# Autodesk Inventor assembly: lift block assy
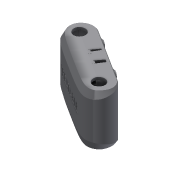
[picture p0: Inventor's stored thumbnail of the model, 180x180]
Saved by Autodesk Inventor 2016 (Build 200138000, 138)
## iProperties
Created: 2016-08-18
Part Number: lift block assy
Document SubType Name: Assembly
Designer: admin
Author: admin
## Documents named in this file (9)
- C:\Users\admin\Desktop\creatablaeD3-이준영 인수인계\1612 3D 도면\lift block assy\lift block assy.iam
- C:\Users\admin\Desktop\creatablaeD3-이준영 인수인계\1612 3D 도면\lift block assy\ball_bushing.ipt
- C:\Users\admin\Desktop\creatablaeD3-이준영 인수인계\1612 3D 도면\lift block assy\belt_fixer.ipt
- C:\Users\admin\Desktop\creatablaeD3-이준영 인수인계\1612 3D 도면\lift block assy\lift_block_cover_back.ipt
- C:\Users\admin\Desktop\creatablaeD3-이준영 인수인계\1612 3D 도면\lift block assy\lift_block_cover_front.ipt
- C:\Users\admin\Desktop\creatablaeD3-이준영 인수인계\1612 3D 도면\lift block assy\m4 15 flat_head_socket.ipt
- C:\Users\admin\Desktop\creatablaeD3-이준영 인수인계\1612 3D 도면\lift block assy\magnet.ipt
- C:\Users\admin\Desktop\creatablaeD3-이준영 인수인계\1612 3D 도면\lift block assy\Ms3 8 BH_tapping_screw.ipt
- C:\Users\admin\Desktop\creatablaeD3-이준영 인수인계\1612 3D 도면\lift block assy\nut_M4.ipt
## Components (13 placed, 8 different names)
1. ball_bushing:1 — Mate:4, Mate:6
2. belt_fixer:1 — Mate:1, Mate:2
3. lift_block_cover_back:1 — Mate:1, Mate:2, Mate:3, Mate:4, Mate:5, Mate:8
4. lift_block_cover_front:1 — Mate:6, Mate:7, Mate:8
5. m4 15 flat_head_socket:1 — Rotational:1, Mate:3
6. magnet:1
7. Ms3 8 BH_tapping_screw:1
8. nut_M4:1 — Rotational:1
9. ball_bushing:2 — Mate:5, Mate:7
10. magnet:2
11. Ms3 8 BH_tapping_screw:2
12. Ms3 8 BH_tapping_screw:3
13. Ms3 8 BH_tapping_screw:4
## Relationships (9: Mate 8, RevoluteJoint 1)
- Mate:1: belt_fixer:1 ↔ lift_block_cover_back:1
- Rotational:1 [RevoluteJoint] (-2 mm): m4 15 flat_head_socket:1 ↔ nut_M4:1
- Mate:2: belt_fixer:1 ↔ lift_block_cover_back:1
- Mate:3: lift_block_cover_back:1 ↔ m4 15 flat_head_socket:1
- Mate:4: ball_bushing:1 ↔ lift_block_cover_back:1
- Mate:5: lift_block_cover_back:1 ↔ ball_bushing:2
- Mate:6: ball_bushing:1 ↔ lift_block_cover_front:1
- Mate:7: lift_block_cover_front:1 ↔ ball_bushing:2
- Mate:8: lift_block_cover_back:1 ↔ lift_block_cover_front:1
